# Autodesk Inventor assembly: ASY MSC 600 cone exit back
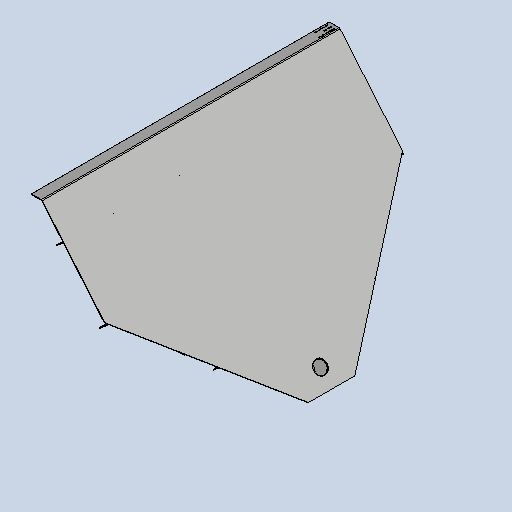
[picture p0: Inventor's stored thumbnail of the model, 512x512]
Saved by Autodesk Inventor 2025 (Build 290162010, 162A)
## iProperties
Created: 2024-08-26
Part Number: ASY MSC 600 cone exit back
Document SubType Name: Assembly
Designer: pokla
Stock Number: ASY МОО 600 конус выход корма
Author: pokla
## Documents named in this file (10)
- C:\Users\pokla\Documents\Inventor\Отстойник осветлитель\Manturovo_Se-clar-Gleb\ASY MSC 600 cone exit back.iam
- C:\Users\pokla\Documents\Inventor\Отстойник осветлитель\Manturovo_Se-clar-Gleb\конус\MSC 601 cone exit back.ipt
- C:\Users\pokla\Documents\Inventor\Отстойник осветлитель\Manturovo_Se-clar-Gleb\конус\MSC 602 stringer cone exit back.ipt
- C:\Users\pokla\Documents\Inventor\Отстойник осветлитель\Manturovo_Se-clar-Gleb\конус\MSC 603 stringer cone exit back.ipt
- C:\Users\pokla\Documents\Inventor\Отстойник осветлитель\Manturovo_Se-clar-Gleb\конус\MSC 604 rib cone exit back.ipt
- C:\Users\pokla\Documents\Inventor\Отстойник осветлитель\Manturovo_Se-clar-Gleb\конус\MSC 605 rib cone exit back.ipt
- C:\Users\pokla\Documents\Inventor\Отстойник осветлитель\Manturovo_Se-clar-Gleb\ракета\MSC 606 rocket tube 6.ipt
- C:\Users\pokla\Documents\Inventor\Отстойник осветлитель\Manturovo_Se-clar-Gleb\ракета\MSC 607 rocket tube 7.ipt
- C:\Users\pokla\Documents\Inventor\Отстойник осветлитель\Manturovo_Se-clar-Gleb\3d party\Stamp flange DIN2642\Stamd flange lapped collar DIN2642\Stamp flange DIN2642-065.ipt
- C:\Users\admin\YandexDisk-badmisterfox\домашниий пк\Inventor\Manturovo\Manturovo_Se-clar\3d party\Stamp flange DIN2642\Stamd flange lapped collar DIN2642.ipt
## Components (11 placed, 8 different names)
1. MSC 016 cone exit back.ipt:1 — Mate:5, Flush:1, Mate:6
2. MSC 0161 stringer cone exit back.ipt:1 — Rigid:5
3. MSC 0161 stringer cone exit back.ipt:2 — Rigid:6
4. MSC 0162 stringer cone exit back.ipt:1 — Rigid:3
5. MSC 0162 stringer cone exit back.ipt:2 — Rigid:4
6. MSC 0163 rib cone exit back.ipt:1 — Mate:5, Flush:1, Mate:6, Rigid:1, Rigid:3, Rigid:4, Rigid:5, Rigid:6
7. MSC 0163 rib cone exit back.ipt:2 — Rigid:1, Rigid:2
8. MSC 0164 rib cone exit back.ipt:1 — Rigid:2
9. МОО 065 ракета труба 5.ipt:1 — Rigid:9
10. МОО 067 ракета труба 7.ipt:1
11. Stamp flange DIN2642-065.ipt:1 — Rigid:9
## Relationships (12: WeldJoint 9, Mate 2, Flush 1)
- Mate:5: MSC 016 cone exit back.ipt:1 ↔ MSC 0163 rib cone exit back.ipt:1
- Flush:1: MSC 016 cone exit back.ipt:1 ↔ MSC 0163 rib cone exit back.ipt:1
- Mate:6 (188.5 mm): MSC 016 cone exit back.ipt:1 ↔ MSC 0163 rib cone exit back.ipt:1
- Rigid:1 [WeldJoint] (374 mm): MSC 0163 rib cone exit back.ipt:1 ↔ MSC 0163 rib cone exit back.ipt:2
- Rigid:2 [WeldJoint] (374 mm): MSC 0163 rib cone exit back.ipt:2 ↔ MSC 0164 rib cone exit back.ipt:1
- Rigid:3 [WeldJoint] (2 mm): MSC 0162 stringer cone exit back.ipt:1 ↔ MSC 0163 rib cone exit back.ipt:1
- Rigid:4 [WeldJoint] (2 mm): MSC 0162 stringer cone exit back.ipt:2 ↔ MSC 0163 rib cone exit back.ipt:1
- Rigid:5 [WeldJoint] (2 mm): MSC 0161 stringer cone exit back.ipt:1 ↔ MSC 0163 rib cone exit back.ipt:1
- Rigid:6 [WeldJoint] (2 mm): MSC 0161 stringer cone exit back.ipt:2 ↔ MSC 0163 rib cone exit back.ipt:1
- [WeldJoint]: MSC 016 cone exit back.ipt:1 ↔ МОО 067 ракета труба 7.ipt:1
- [WeldJoint]: МОО 065 ракета труба 5.ipt:1 ↔ МОО 067 ракета труба 7.ipt:1
- Rigid:9 [WeldJoint]: МОО 065 ракета труба 5.ipt:1 ↔ Stamp flange DIN2642-065.ipt:1
